# Autodesk Inventor assembly: scrumtracker
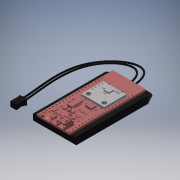
[picture p0: Inventor's stored thumbnail of the model, 180x180]
Saved by Autodesk Inventor 2018 (Build 220112000, 112)
## iProperties
Created: 2018-04-07
Part Number: scrumtracker
Document SubType Name: Assembly
Designer: Raghava
Author: Raghava
## Documents named in this file (4)
- C:\Users\Raghava\Desktop\iot-ball\cad\electronics-subassembly.iam
- C:\Users\Raghava\Desktop\iot-ball\cad\components\esp32-thing.ipt
- C:\Users\Raghava\Desktop\iot-ball\cad\components\li-ion-battery.ipt
- C:\Users\Raghava\Desktop\iot-ball\cad\components\mpu9250-imu.ipt
## Components (3 placed, 3 different names)
1. esp32-thing:1 — Mate:1, Rigid:1, Rigid:2
2. li-ion-battery:1 — Rigid:1
3. mpu9250-imu:1 — Rigid:2
## Relationships (3: WeldJoint 2, Mate 1)
- Mate:1: esp32-thing:1
- Rigid:1 [WeldJoint]: esp32-thing:1 ↔ li-ion-battery:1
- Rigid:2 [WeldJoint] (-4 mm): esp32-thing:1 ↔ mpu9250-imu:1
